# Autodesk Inventor assembly: hurseong
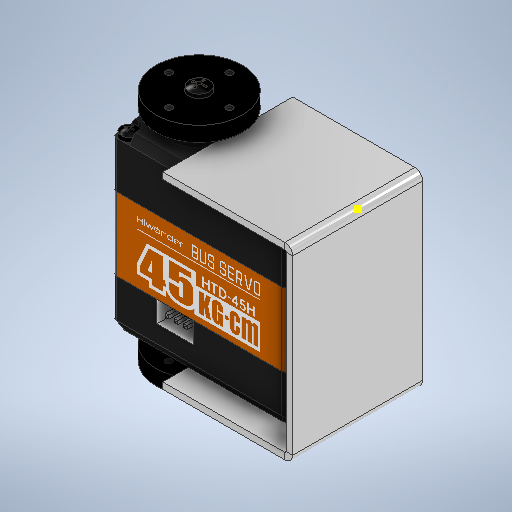
[picture p0: Inventor's stored thumbnail of the model, 512x512]
Saved by Autodesk Inventor 2025.2 (Build 292293000, 293)
## iProperties
Created: 2025-03-25
Part Number: hurseong
Document SubType Name: Assembly
Designer: LG
Author: LG
## Documents named in this file (3)
- C:\Users\LG\Desktop\RHp_hardware_example\Assembly\hurseong.iam
- C:\Users\LG\Desktop\RHp_hardware_example\Part\HTD-45H, Horn\HTD-45H Assembly.iam
- C:\Users\LG\Desktop\RHp_hardware_example\Part\Frame\hurseong.ipt
## Components (2 placed, 2 different names)
1. HTD-45H Assembly:1 [sub-assembly] — Flush:1, Flush:2, Flush:3, Mate:1, Mate:2, Mate:3
2. hurseong:1 — Mate:1, Mate:2, Mate:3
## Relationships (6: Flush 3, Mate 3)
- Flush:1: HTD-45H Assembly:1
- Flush:2: HTD-45H Assembly:1
- Flush:3: HTD-45H Assembly:1
- Mate:1: HTD-45H Assembly:1 ↔ hurseong:1
- Mate:2: HTD-45H Assembly:1 ↔ hurseong:1
- Mate:3 (5 mm): HTD-45H Assembly:1 ↔ hurseong:1
